# Autodesk Inventor assembly: HarmonicDrive
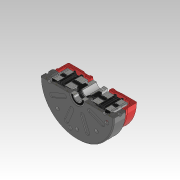
[picture p0: Inventor's stored thumbnail of the model, 180x180]
Saved by Autodesk Inventor 2020 (Build 240168000, 168)
## iProperties
Created: 2021-03-19
Part Number: HarmonicDrive
Document SubType Name: Assembly
Designer: DDeGo
Author: DDeGo
## Documents named in this file (11)
- C:\Users\DDeGo\Documents\Drew\Projects\OS-ARM\cad\HarmonicDrive75mm V2\HarmonicDrive75mmV2.iam
- C:\Users\DDeGo\Documents\Drew\Projects\OS-ARM\cad\HarmonicDrive75mm V2\HD_housing.ipt
- C:\Users\DDeGo\Documents\Drew\Projects\OS-ARM\cad\HarmonicDrive75mm V2\HD_rotor.ipt
- C:\Users\DDeGo\Documents\Drew\Projects\OS-ARM\cad\OTS\Radial Bearings\608 bearing.ipt
- C:\Users\DDeGo\Documents\Drew\Projects\OS-ARM\cad\HarmonicDrive75mm V2\HD_housing2.ipt
- C:\Users\DDeGo\Documents\Drew\Projects\OS-ARM\cad\HarmonicDrive75mm V2\HD_BearingShaft1.ipt
- C:\Users\DDeGo\Documents\Drew\Projects\OS-ARM\cad\HarmonicDrive75mm V2\HD_BearingShaft2.ipt
- C:\Users\DDeGo\Documents\Drew\Projects\OS-ARM\cad\HarmonicDrive75mm V2\HD_rotorshim.ipt
- C:\Users\DDeGo\Documents\Drew\Projects\OS-ARM\cad\OTS\Radial Bearings\688 bearing.ipt
- C:\Users\DDeGo\Documents\Drew\Projects\OS-ARM\cad\HarmonicDrive75mm V2\HD_FlexSpline_involute_205_15.ipt
- C:\Users\DDeGo\Documents\Drew\Projects\OS-ARM\cad\OTS\Other\GT2Pulley_20T_8mm_noTop.ipt
## Components (18 placed, 10 different names)
1. HD_housing:1 — Mate:53, Mate:54, Mate:57, Mate:60, Angle:1, Mate:63, Mate:64
2. HD_rotor:1 — Mate:4, Mate:5, Mate:9, Mate:11, Mate:65, Mate:66, Mate:67, Mate:68, Mate:69, Mate:70, Mate:71, Flush:1, Rotation:1
3. HD_housing2:1 — Mate:53, Mate:60, Angle:1, Rotation:1
4. 608 bearing:2 — Mate:5, Mate:34, Mate:38, Mate:47
5. 608 bearing:3 — Mate:4, Mate:36, Mate:39, Mate:48
6. 608 bearing:5 — Mate:9, Mate:33, Mate:37, Mate:51
7. 608 bearing:6 — Mate:11, Mate:35, Mate:40, Mate:52
8. HD_BearingShaft1:1 — Mate:35, Mate:40
9. HD_BearingShaft2:1 — Mate:33, Mate:37, Mate:41, Mate:42
10. HD_BearingShaft1:2 — Mate:36, Mate:39
11. HD_BearingShaft2:2 — Mate:34, Mate:38, Mate:43, Mate:44
12. HD_rotorshim:1 — Mate:41, Mate:51, Mate:67
13. HD_rotorshim:2 — Mate:42, Mate:52, Mate:68
14. HD_rotorshim:3 — Mate:43, Mate:47, Mate:66
15. HD_rotorshim:4 — Mate:44, Mate:48, Mate:69
16. 688 bearing:1 — Mate:54, Mate:57, Mate:65, Mate:72
17. HD_FlexSpline_involute_205_15:1 — Mate:63, Mate:64
18. GT2Pulley_20T_8mm_noTop:1 — Mate:70, Mate:71, Mate:72, Flush:1
## Relationships (37: Mate 34, Angle 1, Flush 1, RelateRotation 1)
- Mate:4: HD_rotor:1 ↔ 608 bearing:3
- Mate:5: HD_rotor:1 ↔ 608 bearing:2
- Mate:9: HD_rotor:1 ↔ 608 bearing:5
- Mate:11: HD_rotor:1 ↔ 608 bearing:6
- Mate:33: 608 bearing:5 ↔ HD_BearingShaft2:1
- Mate:34: 608 bearing:2 ↔ HD_BearingShaft2:2
- Mate:35: 608 bearing:6 ↔ HD_BearingShaft1:1
- Mate:36: 608 bearing:3 ↔ HD_BearingShaft1:2
- Mate:37: 608 bearing:5 ↔ HD_BearingShaft2:1
- Mate:38: 608 bearing:2 ↔ HD_BearingShaft2:2
- Mate:39: 608 bearing:3 ↔ HD_BearingShaft1:2
- Mate:40: 608 bearing:6 ↔ HD_BearingShaft1:1
- Mate:41: HD_BearingShaft2:1 ↔ HD_rotorshim:1
- Mate:42: HD_BearingShaft2:1 ↔ HD_rotorshim:2
- Mate:43: HD_BearingShaft2:2 ↔ HD_rotorshim:3
- Mate:44: HD_BearingShaft2:2 ↔ HD_rotorshim:4
- Mate:47: 608 bearing:2 ↔ HD_rotorshim:3
- Mate:48: 608 bearing:3 ↔ HD_rotorshim:4
- Mate:51: 608 bearing:5 ↔ HD_rotorshim:1
- Mate:52: 608 bearing:6 ↔ HD_rotorshim:2
- Mate:53 (1 mm): HD_housing:1 ↔ HD_housing2:1
- Mate:54: HD_housing:1 ↔ 688 bearing:1
- Mate:57: HD_housing:1 ↔ 688 bearing:1
- Mate:60: HD_housing:1 ↔ HD_housing2:1
- Angle:1 (0 deg): HD_housing:1 ↔ HD_housing2:1
- Mate:63: HD_housing:1 ↔ HD_FlexSpline_involute_205_15:1
- Mate:64: HD_housing:1 ↔ HD_FlexSpline_involute_205_15:1
- Mate:65: HD_rotor:1 ↔ 688 bearing:1
- Mate:66: HD_rotor:1 ↔ HD_rotorshim:3
- Mate:67: HD_rotor:1 ↔ HD_rotorshim:1
- Mate:68: HD_rotor:1 ↔ HD_rotorshim:2
- Mate:69: HD_rotor:1 ↔ HD_rotorshim:4
- Mate:70: HD_rotor:1 ↔ GT2Pulley_20T_8mm_noTop:1
- Mate:71: HD_rotor:1 ↔ GT2Pulley_20T_8mm_noTop:1
- Mate:72: 688 bearing:1 ↔ GT2Pulley_20T_8mm_noTop:1
- Flush:1: HD_rotor:1 ↔ GT2Pulley_20T_8mm_noTop:1
- Rotation:1 [RelateRotation] (34 ul): HD_rotor:1 ↔ HD_housing2:1
